# Autodesk Inventor assembly: LowerBody
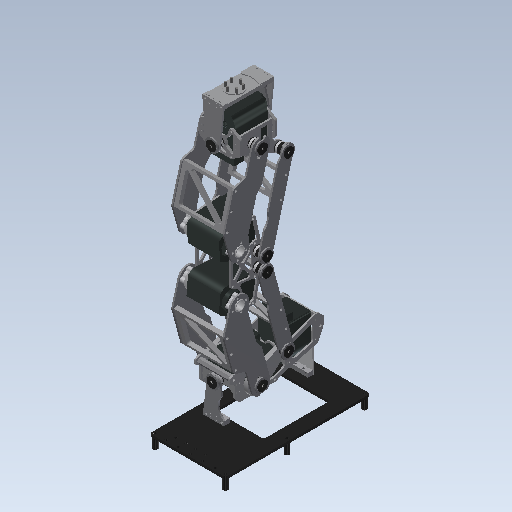
[picture p0: Inventor's stored thumbnail of the model, 512x512]
Saved by Autodesk Inventor 2020.4 (Build 244396000, 396)
## iProperties
Created: 2016-08-23
Part Number: LowerBody
Material: 一般
Document SubType Name: Assembly
Designer: hiro
Mass: 988.92 g
Surface Area: 2590.63 cm^2
Volume: 450.085 cm^3
Density: 2.19718 g/cm^3
Author: hiro
## Documents named in this file (13)
- C:\Users\Masato\Documents\Inventor\CIT Brains_Inventor\OpenPlatform_ver3_0\LowerBody.iam
- C:\Users\Masato\Documents\Inventor\CIT Brains_Inventor\OpenPlatform_ver3_0\LowerBody\Ankle\Ankle.iam
- C:\Users\Masato\Documents\Inventor\CIT Brains_Inventor\OpenPlatform_ver3_0\LowerBody\Ankle\Ankle_side_pitch.iam
- C:\Users\Masato\Documents\Inventor\CIT Brains_Inventor\OpenPlatform_ver3_0\LowerBody\Link\LowerFrontLink.iam
- C:\Users\Masato\Documents\Inventor\CIT Brains_Inventor\OpenPlatform_ver3_0\LowerBody\Leg_joint_roll\Leg_Joint_roll.iam
- C:\Users\Masato\Documents\Inventor\CIT Brains_Inventor\OpenPlatform_ver3_0\LowerBody\Link\LowerBackLink.iam
- C:\Users\Masato\Documents\Inventor\CIT Brains_Inventor\OpenPlatform_ver3_0\LowerBody\Slider_crank\Slider_crank_mechanism.iam
- C:\Users\Masato\Documents\Inventor\CIT Brains_Inventor\OpenPlatform_ver3_0\LowerBody\Knee\Knee.iam
- C:\Users\Masato\Documents\Inventor\CIT Brains_Inventor\OpenPlatform_ver3_0\LowerBody\Leg_joit\Leg_joint.iam
- C:\Users\Masato\Documents\Inventor\CIT Brains_Inventor\OpenPlatform_ver3_0\LowerBody\Link\UpperBackLink.iam
- C:\Users\Masato\Documents\Inventor\CIT Brains_Inventor\OpenPlatform_ver3_0\LowerBody\Link\UpperFrontLink.iam
- C:\Users\Masato\Documents\Inventor\CIT Brains_Inventor\OpenPlatform_ver3_0\LowerBody\Foot\foot.iam
- C:\Users\Masato\Documents\Inventor\CIT Brains_Inventor\OpenPlatform_ver3_0\Ready_Made\Screw\M2_5-10.ipt
## Components (18 placed, 12 different names)
1. 付け根ロール_1:1 [sub-assembly] — 角度:12, 挿入:146, 挿入:147, 角度:14, 挿入:153, 挿入:154, 挿入:155, 挿入:156, 挿入:157, 挿入:158
2. Slider_crank_mechanism:1 [sub-assembly] — 挿入:145, 挿入:146
3. 付け根_1:1 [sub-assembly] — メイト:1, メイト:2, 挿入:142, 挿入:144, 挿入:145, 挿入:147
4. UpperFrontLink:1 [sub-assembly] — 角度:12, 挿入:139, 挿入:144
5. UpperBackLink:1 [sub-assembly] — 挿入:141, 挿入:142
6. 膝_1:1 [sub-assembly] — 挿入:129, 挿入:139, 挿入:141, 挿入:143
7. LowerFrontLink:2 [sub-assembly] — 挿入:129, 挿入:148, 角度:13
8. LowerBackLink:1 [sub-assembly] — 挿入:143, 挿入:149, 挿入:151
9. 足首_1:1 [sub-assembly] — 挿入:124, 挿入:150, 挿入:152
10. Foot:1 [sub-assembly] — 挿入:152, 角度:13, 角度:14
11. 足首_独立ピッチ_1:1 [sub-assembly] — 挿入:124, 挿入:148, 挿入:149
12. 足首_独立ピッチ_1:2 [sub-assembly] — 挿入:150, 挿入:151
13. M2_5-10:1 — 挿入:153
14. M2_5-10:2 — 挿入:154
15. M2_5-10:3 — 挿入:155
16. M2_5-10:4 — 挿入:156
17. M2_5-10:5 — 挿入:157
18. M2_5-10:6 — 挿入:158
## Relationships (26: Insert 21, Angle 3, Mate 2)
- 角度:12 [Angle] (15 deg): 付け根ロール_1:1 ↔ UpperFrontLink:1
- 挿入:124 [Insert]: 足首_1:1 ↔ 足首_独立ピッチ_1:1
- 挿入:129 [Insert]: 膝_1:1 ↔ LowerFrontLink:2
- メイト:1 [Mate] (-16.5 mm): 付け根_1:1
- メイト:2 [Mate] (-27 mm): 付け根_1:1
- 挿入:139 [Insert]: UpperFrontLink:1 ↔ 膝_1:1
- 挿入:141 [Insert]: UpperBackLink:1 ↔ 膝_1:1
- 挿入:142 [Insert]: 付け根_1:1 ↔ UpperBackLink:1
- 挿入:143 [Insert]: 膝_1:1 ↔ LowerBackLink:1
- 挿入:144 [Insert]: 付け根_1:1 ↔ UpperFrontLink:1
- 挿入:145 [Insert]: Slider_crank_mechanism:1 ↔ 付け根_1:1
- 挿入:146 [Insert]: 付け根ロール_1:1 ↔ Slider_crank_mechanism:1
- 挿入:147 [Insert]: 付け根ロール_1:1 ↔ 付け根_1:1
- 挿入:148 [Insert]: LowerFrontLink:2 ↔ 足首_独立ピッチ_1:1
- 挿入:149 [Insert]: LowerBackLink:1 ↔ 足首_独立ピッチ_1:1
- 挿入:150 [Insert]: 足首_1:1 ↔ 足首_独立ピッチ_1:2
- 挿入:151 [Insert]: LowerBackLink:1 ↔ 足首_独立ピッチ_1:2
- 挿入:152 [Insert]: 足首_1:1 ↔ Foot:1
- 角度:13 [Angle] (15 deg): LowerFrontLink:2 ↔ Foot:1
- 角度:14 [Angle] (0 deg): 付け根ロール_1:1 ↔ Foot:1
- 挿入:153 [Insert]: 付け根ロール_1:1 ↔ M2_5-10:1
- 挿入:154 [Insert]: 付け根ロール_1:1 ↔ M2_5-10:2
- 挿入:155 [Insert]: 付け根ロール_1:1 ↔ M2_5-10:3
- 挿入:156 [Insert]: 付け根ロール_1:1 ↔ M2_5-10:4
- 挿入:157 [Insert]: 付け根ロール_1:1 ↔ M2_5-10:5
- 挿入:158 [Insert]: 付け根ロール_1:1 ↔ M2_5-10:6
